# Autodesk Inventor assembly: ShoulderConnectorSplit
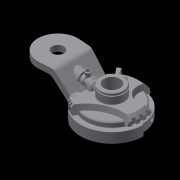
[picture p0: Inventor's stored thumbnail of the model, 180x180]
Saved by Autodesk Inventor 2015 (Build 190159000, 159)
## iProperties
Created: 2015-12-02
Part Number: ShoulderConnectorSplit
Document SubType Name: Assembly
Designer: Val
Author: Val
## Documents named in this file (3)
- D:\Desktop\ExoBackup8\ShoulderConnectorSplit.iam
- D:\Desktop\ExoBackup8\ShoulderConnectorSplitBody.ipt
- D:\Desktop\ExoBackup8\ShoulderConnectorSplitHead.ipt
## Components (2 placed, 2 different names)
1. ShoulderConnectorSplitBody:1 — Mate:1, Mate:2
2. ShoulderConnectorSplitHead:1 — Mate:1, Mate:2
## Relationships (2: Mate 2)
- Mate:1: ShoulderConnectorSplitBody:1 ↔ ShoulderConnectorSplitHead:1
- Mate:2: ShoulderConnectorSplitBody:1 ↔ ShoulderConnectorSplitHead:1
